# Autodesk Inventor assembly: Assy_fork_right
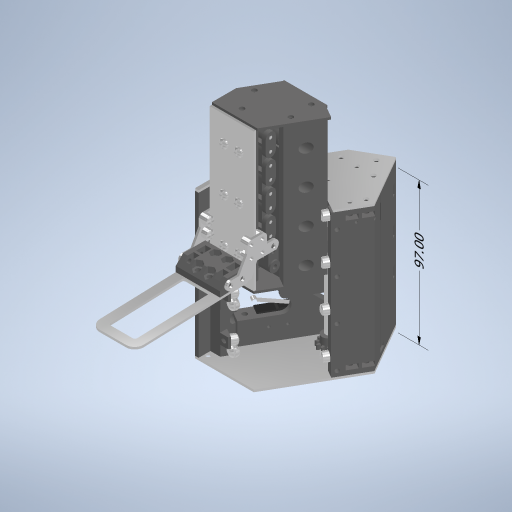
[picture p0: Inventor's stored thumbnail of the model, 512x512]
Saved by Autodesk Inventor 2024.1 (Build 281209000, 209)
## iProperties
Created: 2025-01-17
Part Number: Assy_fork_right
Document SubType Name: Assembly
Designer: hibik
Author: hibik
## Documents named in this file (7)
- C:\Users\hibik\Documents\Robomech\RESCUE\ORCA\hard\fork\right\Assy_fork_right.iam
- C:\Users\hibik\Documents\Robomech\RESCUE\ORCA\hard\fork\right\base_wall_added.iam
- C:\Users\hibik\Documents\Robomech\RESCUE\ORCA\hard\fork\right\motor_set.iam
- C:\Users\hibik\Documents\Robomech\RESCUE\ORCA\hard\fork\right\screw_middle_gear_under_12.ipt
- C:\Users\hibik\Documents\Robomech\RESCUE\ORCA\hard\fork\right\screw.iam
- C:\Users\hibik\Documents\Robomech\RESCUE\ORCA\hard\board\CORE_model\md.iam
- C:\Users\hibik\Documents\Robomech\RESCUE\ORCA\hard\fork\right\rail.iam
## Components (6 placed, 6 different names)
1. motor_set:1 [sub-assembly] — 挿入:5, 角度:1
2. screw_middle_gear_under_12:1 — 挿入:6
3. base_wall_added:1 [sub-assembly] — 挿入:3, フラッシュ:1, 挿入:4, 挿入:5, 角度:1, 挿入:6, 正接:1, 正接:2, 正接:3
4. screw:1 [sub-assembly] — 挿入:3
5. md:1 [sub-assembly] — フラッシュ:1, 挿入:4
6. rail:1 [sub-assembly] — 正接:1, 正接:2, 正接:3
## Relationships (9: Insert 4, Tangent 3, Flush 1, Angle 1)
- 挿入:3 [Insert]: base_wall_added:1 ↔ screw:1
- フラッシュ:1 [Flush]: base_wall_added:1 ↔ md:1
- 挿入:4 [Insert]: base_wall_added:1 ↔ md:1
- 挿入:5 [Insert]: motor_set:1 ↔ base_wall_added:1
- 角度:1 [Angle] (0 deg): motor_set:1 ↔ base_wall_added:1
- 挿入:6 [Insert]: screw_middle_gear_under_12:1 ↔ base_wall_added:1
- 正接:1 [Tangent]: base_wall_added:1 ↔ rail:1
- 正接:2 [Tangent]: base_wall_added:1 ↔ rail:1
- 正接:3 [Tangent]: base_wall_added:1 ↔ rail:1
